# Autodesk Inventor assembly: Forearm
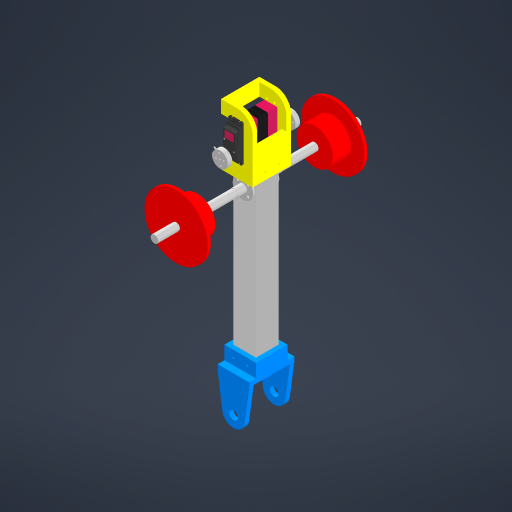
[picture p0: Inventor's stored thumbnail of the model, 512x512]
Saved by Autodesk Inventor 2023 (Build 270158000, 158)
## iProperties
Created: 2023-08-18
Part Number: Forearm
Document SubType Name: Assembly
Designer: Abhinav
Author: Abhinav
## Documents named in this file (9)
- C:\Users\Abhinav\Desktop\GRID\ARM 3\Forearm\00_Forearm.iam
- C:\Users\Abhinav\Desktop\3D Library\60 kg cm Servo.ipt
- C:\Users\Abhinav\Desktop\GRID\ARM 3\Forearm\Joint_3_House.ipt
- C:\Users\Abhinav\Desktop\GRID\ARM 3\Forearm\Forearm-Link.ipt
- C:\Users\Abhinav\Desktop\GRID\ARM 3\Forearm\Forearm-End Fork.ipt
- C:\Users\Abhinav\Desktop\GRID\ARM 3\Forearm\Pulley-35.ipt
- C:\Users\Abhinav\Desktop\GRID\ARM 3\Forearm\Forearm-Shaft.ipt
- C:\Users\Abhinav\Desktop\GRID\ARM 3\Forearm\12mm Flange.ipt
- C:\Users\Abhinav\Desktop\GRID\ARM 3\Forearm\47T-Sprocket.ipt
## Components (12 placed, 8 different names)
1. 60 kg cm Servo:1 — Mate:7, Mate:8, Mate:9, Mate:21
2. 60 kg cm Servo:2 — Mate:10, Mate:11, Mate:12, Mate:23
3. Joint_3_House:1 — Mate:7, Mate:8, Mate:9, Mate:10, Mate:11, Mate:12, Mate:14, Mate:15, Mate:19
4. Forearm-Link:1 — Mate:14, Mate:15, Mate:16, Mate:17, Mate:18, Mate:19, Flush:2, Mate:26, Mate:30, Mate:31, Mate:32, Mate:33, Mate:34, Mate:20, Mate:22, Flush:3, Flush:4
5. Forearm-End Fork:1 — Mate:16, Mate:17, Mate:18
6. Pulley-35:1 — Mate:20, Mate:21, Flush:1
7. Pulley-35:2 — Mate:22, Mate:23, Flush:1
8. Forearm-Shaft:1 — Flush:2, Mate:25, Mate:28, Mate:35, Mate:36
9. 12mm Flange:1 — Mate:25, Mate:26, Mate:33, Mate:34
10. 12mm Flange:2 — Mate:28, Mate:30, Mate:31, Mate:32
11. 47T-Sprocket:1 — Mate:35, Flush:3
12. 47T-Sprocket:2 — Mate:36, Flush:4
## Relationships (30: Mate 26, Flush 4)
- Mate:7: 60 kg cm Servo:1 ↔ Joint_3_House:1
- Mate:8: 60 kg cm Servo:1 ↔ Joint_3_House:1
- Mate:9: 60 kg cm Servo:1 ↔ Joint_3_House:1
- Mate:10: 60 kg cm Servo:2 ↔ Joint_3_House:1
- Mate:11: 60 kg cm Servo:2 ↔ Joint_3_House:1
- Mate:12: 60 kg cm Servo:2 ↔ Joint_3_House:1
- Mate:14 (7.5 mm): Joint_3_House:1 ↔ Forearm-Link:1
- Mate:15: Joint_3_House:1 ↔ Forearm-Link:1
- Mate:16: Forearm-Link:1 ↔ Forearm-End Fork:1
- Mate:17: Forearm-Link:1 ↔ Forearm-End Fork:1
- Mate:18: Forearm-Link:1 ↔ Forearm-End Fork:1
- Mate:19: Joint_3_House:1 ↔ Forearm-Link:1
- Mate:20 (45 mm): Forearm-Link:1 ↔ Pulley-35:1
- Mate:21: 60 kg cm Servo:1 ↔ Pulley-35:1
- Mate:22 (45 mm): Forearm-Link:1 ↔ Pulley-35:2
- Mate:23: 60 kg cm Servo:2 ↔ Pulley-35:2
- Flush:1: Pulley-35:1 ↔ Pulley-35:2
- Flush:2 (-200 mm): Forearm-Link:1 ↔ Forearm-Shaft:1
- Mate:25: Forearm-Shaft:1 ↔ 12mm Flange:1
- Mate:26: Forearm-Link:1 ↔ 12mm Flange:1
- Mate:28: Forearm-Shaft:1 ↔ 12mm Flange:2
- Mate:30: Forearm-Link:1 ↔ 12mm Flange:2
- Mate:31: Forearm-Link:1 ↔ 12mm Flange:2
- Mate:32: Forearm-Link:1 ↔ 12mm Flange:2
- Mate:33: Forearm-Link:1 ↔ 12mm Flange:1
- Mate:34: Forearm-Link:1 ↔ 12mm Flange:1
- Mate:35: Forearm-Shaft:1 ↔ 47T-Sprocket:1
- Flush:3 (-152 mm): Forearm-Link:1 ↔ 47T-Sprocket:1
- Mate:36: Forearm-Shaft:1 ↔ 47T-Sprocket:2
- Flush:4 (152 mm): Forearm-Link:1 ↔ 47T-Sprocket:2
